# Autodesk Inventor assembly: Z Belt Clip with HSI
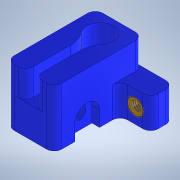
[picture p0: Inventor's stored thumbnail of the model, 180x180]
Saved by Autodesk Inventor 2022 (Build 260153000, 153)
## iProperties
Created: 2022-03-21
Part Number: Z Belt Clip with HSI
Document SubType Name: Assembly
Designer: Nick
Author: Nick
## Documents named in this file (3)
- Y:\Projects\Bibble0\3D printed\Z Axis\Z Belt Tensioner HSI.iam
- Y:\Projects\Bibble0\3D printed\Z Axis\Z Belt Tensioner.ipt
- Y:\Projects\Bibble0\Hardware\M3 Heat Set Inserts.ipt
## Components (3 placed, 2 different names)
1. Z Belt Tensioner:1 — Insert:1, Insert:2
2. M3 Heat Set Inserts:1 — Insert:1
3. M3 Heat Set Inserts:2 — Insert:2
## Relationships (2: Insert 2)
- Insert:1: Z Belt Tensioner:1 ↔ M3 Heat Set Inserts:1
- Insert:2: Z Belt Tensioner:1 ↔ M3 Heat Set Inserts:2
